# Autodesk Inventor assembly: switchblade
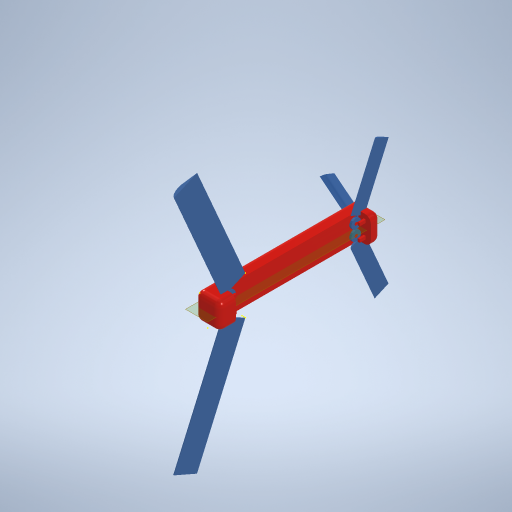
[picture p0: Inventor's stored thumbnail of the model, 512x512]
Saved by Autodesk Inventor 2023 (Build 270158000, 158)
## iProperties
Created: 2023-05-23
Part Number: switchblade
Document SubType Name: Assembly
Designer: Sujeet Kumar
Author: Sujeet Kumar
## Documents named in this file (7)
- C:\Users\Sujeet Kumar\Desktop\switchblade V1\switchblade.iam
- C:\Users\Sujeet Kumar\Desktop\switchblade V1\plane body.ipt
- C:\Users\Sujeet Kumar\Desktop\switchblade V1\R wing.ipt
- C:\Users\Sujeet Kumar\Desktop\switchblade V1\R wing_MIR.ipt
- C:\Users\Sujeet Kumar\Desktop\switchblade V1\elevator.ipt
- C:\Users\Sujeet Kumar\Desktop\switchblade V1\elevator_MIR.ipt
- C:\Users\Sujeet Kumar\Desktop\switchblade V1\Ruder.ipt
## Components (6 placed, 6 different names)
1. plane body:1 — Mate:1, Mate:2, Mate:3, Mate:4, Mate:5, Mate:6, Mate:7, Mate:8, Mate:9, Mate:10
2. R wing:1 — Mate:1, Mate:2, Rotation:1, Rotation:3
3. R wing_MIR:1 — Mate:3, Mate:4, Rotation:1
4. elevator:1 — Mate:5, Mate:6, Rotation:2, Rotation:3, Rotation:4
5. elevator_MIR:1 — Mate:7, Mate:8, Rotation:2
6. Ruder:1 — Mate:9, Mate:10, Rotation:4
## Relationships (14: Mate 10, RelateRotation 4)
- Mate:1: plane body:1 ↔ R wing:1
- Mate:2 (2 mm): plane body:1 ↔ R wing:1
- Mate:3: plane body:1 ↔ R wing_MIR:1
- Mate:4 (2 mm): plane body:1 ↔ R wing_MIR:1
- Mate:5: plane body:1 ↔ elevator:1
- Mate:6 (2 mm): plane body:1 ↔ elevator:1
- Mate:7: plane body:1 ↔ elevator_MIR:1
- Mate:8 (2 mm): plane body:1 ↔ elevator_MIR:1
- Rotation:1 [RelateRotation] (1 ul): R wing:1 ↔ R wing_MIR:1
- Rotation:2 [RelateRotation] (1 ul): elevator:1 ↔ elevator_MIR:1
- Rotation:3 [RelateRotation] (1 ul): R wing:1 ↔ elevator:1
- Mate:9: plane body:1 ↔ Ruder:1
- Mate:10: plane body:1 ↔ Ruder:1
- Rotation:4 [RelateRotation] (1 ul): elevator:1 ↔ Ruder:1
